# Autodesk Inventor assembly: Generic_Pillow_Block
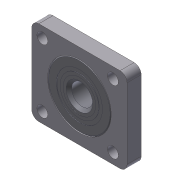
[picture p0: Inventor's stored thumbnail of the model, 180x180]
Saved by Autodesk Inventor 2012 (Build 160160000, 160)
## iProperties
Created: 2012-01-29
Part Number: Generic_Pillow_Block
Document SubType Name: Assembly
Designer: JesseK
Mass: 55.5579 g
Surface Area: 92.9614 cm^2
Volume: 10.7096 cm^3
Density: 5.18768 g/cm^3
Author: JesseK
## Documents named in this file (3)
- Z:\UserData\Documents\Inventor\team1885frc\Robot2012\Misc\Generic_Pillow_Block.iam
- Z:\UserData\Documents\Inventor\team1885frc\Robot2012\Misc\Generic_Pillow_Block.ipt
- Z:\UserData\Documents\Inventor\team1885frc\Hardware\Bearings\Bearing_0.375ID_1.125OD.ipt
## Components (2 placed, 2 different names)
1. Generic_Pillow_Block:1 — Flush:1, Mate:1
2. Bearing_0.375ID_1.125OD:1 — Flush:1, Mate:1
## Relationships (2: Flush 1, Mate 1)
- Flush:1: Generic_Pillow_Block:1 ↔ Bearing_0.375ID_1.125OD:1
- Mate:1: Generic_Pillow_Block:1 ↔ Bearing_0.375ID_1.125OD:1
